# Autodesk Inventor assembly: Finger Mold 2
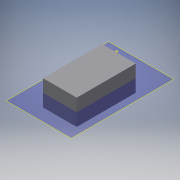
[picture p0: Inventor's stored thumbnail of the model, 180x180]
Saved by Autodesk Inventor 2016 (Build 200138000, 138)
## iProperties
Created: 2015-06-26
Part Number: Finger Mold 2
Document SubType Name: Assembly
Designer: Jack
Author: Jack
## Documents named in this file (3)
- D:\Autodesk Inventor\Finger Mold 2.iam
- D:\Autodesk Inventor\Finger Mold.ipt
- D:\Autodesk Inventor\Full Rubber Finger.ipt
## Components (3 placed, 2 different names)
1. Finger Mold:1 — Mate:1, Mate:2, Mate:3, Mate:4
2. Finger Mold:2 — Mate:2, Mate:3, Mate:4
3. Full Rubber Finger:1 — Mate:1
## Relationships (4: Mate 4)
- Mate:1: Finger Mold:1 ↔ Full Rubber Finger:1
- Mate:2: Finger Mold:1 ↔ Finger Mold:2
- Mate:3: Finger Mold:1 ↔ Finger Mold:2
- Mate:4: Finger Mold:1 ↔ Finger Mold:2
